# Autodesk Inventor assembly: ASY TZS 1240 FDS Top elbow
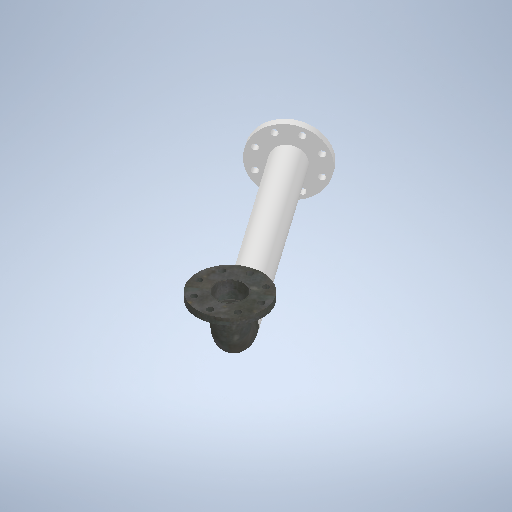
[picture p0: Inventor's stored thumbnail of the model, 512x512]
Saved by Autodesk Inventor 2025 (Build 290162010, 162A)
## iProperties
Created: 2025-07-10
Part Number: ASY TZS 1240 FDS Top elbow
Document SubType Name: Assembly
Designer: user
Author: user
## Documents named in this file (5)
- C:\Users\pokla\Documents\Inventor\TZS-Tazovskiy\Фильтр D1200\ASY TZS 1240 FDS Top elbow.iam
- C:\Users\pokla\Documents\Inventor\TZS-Tazovskiy\Фильтр D1200\DIN 2576 Slip-On Flange for Welding Series 1 (ISO) - PN 10 80 x 88.9.ipt
- C:\Users\pokla\Documents\Inventor\TZS-Tazovskiy\Фильтр D1200\TZS 1242 FDS  tube 1.ipt
- C:\Users\pokla\Documents\Inventor\TZS-Tazovskiy\Фильтр D1200\TZS 1241 FDS tube 1.ipt
- C:\Users\pokla\Documents\Inventor\Content Center Files\R2025\en-US\JIS B 2312 90 (2)\JIS B 2312 90 Deg Long Elbow Steel 80A x Sch 40.ipt
## Components (5 placed, 4 different names)
1. DIN 2576 Slip-On Flange for Welding Series 1 (ISO) - PN 10 80 x 88.9.ipt:1 — Rigid:7
2. TZS 1241 FDS tube 1.ipt:1 — Rigid:7
3. JIS B 2312 90 Deg Long Elbow Steel 100A x Sch 40.ipt:1
4. TZS 1242 FDS  tube 1.ipt:1
5. DIN 2576 Slip-On Flange for Welding Series 1 (ISO) - PN 10 80 x 88.9.ipt:2
## Relationships (4: WeldJoint 4)
- [WeldJoint]: TZS 1241 FDS tube 1.ipt:1 ↔ JIS B 2312 90 Deg Long Elbow Steel 100A x Sch 40.ipt:1
- [WeldJoint]: JIS B 2312 90 Deg Long Elbow Steel 100A x Sch 40.ipt:1 ↔ TZS 1242 FDS  tube 1.ipt:1
- [WeldJoint]: TZS 1242 FDS  tube 1.ipt:1 ↔ DIN 2576 Slip-On Flange for Welding Series 1 (ISO) - PN 10 80 x 88.9.ipt:2
- Rigid:7 [WeldJoint]: DIN 2576 Slip-On Flange for Welding Series 1 (ISO) - PN 10 80 x 88.9.ipt:1 ↔ TZS 1241 FDS tube 1.ipt:1
